# Autodesk Inventor assembly: 043-DP
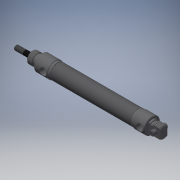
[picture p0: Inventor's stored thumbnail of the model, 180x180]
Saved by Autodesk Inventor 2016 (Build 200138000, 138)
## iProperties
Category: PARTsolutions
Company: BIMBA
Created: 2016-01-18
Part Number: 043-DP
Catalog Web Link: www.cadenas.de
Description: Original Line Standard Air Cylinders-
Vendor: BIMBA
Document SubType Name: Assembly
Designer: psAdmin
Manufacturer: BIMBA
PSOL_IDENT_0: {$CADENAS_DATA\23d-libs\bimba\bimba\bimba_imperial\bimba_full_line\original_line_cylinders\standard_
PSOL_IDENT_1: air_cylinders\standard_air_cylinder_asmtab.prj},312 {VTYP=3D},{STYP=ASSTAB},{NB=043-DP},{LINA=043-DP
PSOL_IDENT_2: },{NN=Original Line Standard Air Cylinders},{DATE=02.12.2015 13:51:22},{GEOMDATE=02.12.2015 13:51:20
PSOL_IDENT_3: },{VERSION=},{LINEID=50},{LINESUBID=-1},{WBVAR=STROKE,ACTING,MNT,DER,NR,BM,CO,OO,VO,M,EE,EEL,K,Q,Y,G
PSOL_IDENT_4: ,T,B,H,SER,SR,NT,W,HL,STPT1,STPT2,STPT3,STPT4,MB,PB,PRC,TB,MN}  {NB=043-DP},{LINA=043-DP},{KT=DUMMY}
PSOL_IDENT_5: ,{PN=043-DP},{PNC=043-DP},{PNA=(NO ACCESSORIES)},{DASH=-},{BORE1=0.75000000},{BORE=3/4\" (04)},{BORE
PSOL_IDENT_6: PN=04},{STROKE=3.000},{STROKEALG=[0.011:50/0.001]},{STROKE1=3.000},{ACTING=D},{ACTINGALG= '' , 'Sing
PSOL_IDENT_7: le Acting (SA)' , 'R' , 'Reverse Single Acting (SA)' , 'D' , 'Double Acting (SA)' },{ACTINGPN=D},{MN
PSOL_IDENT_8: T=P},{MNTALG= '' , 'Front Nose Mounting (SA)' , 'P' , 'Rear Pivot Mounting (SA)' , 'XP' , 'Double En
PSOL_IDENT_9: d or Pivot Mounting (SA)' , 'X' , 'Double End Mounting (SA)' , 'BF' , 'Front Block Mounting (SA)' , '
PSOL_IDENT_10: BR' , 'Rear Block Mounting for Vertical Positioning (SA)' , 'BFT' , 'Front Block Trunnion Mounting (
PSOL_IDENT_11: SA)' , 'BRT' , 'Rear Block Trunnion Mounting (SA)' },{TYPE=},{MNTPN=P},{DER=},{DERALG= '' , 'N/A' },
PSOL_IDENT_12: {NR=},{NRALG= '' , 'N/A' },{NRPN=},{BM=},{BMALG= '' , 'N/A' },{BMPN=},{CO=},{COALG= '' , 'N/A' },{OO=
PSOL_IDENT_13: },{OOALG= '', 'N/A' },{OOPN=},{VO=Z},{VOALG= 'Z' , 'N/A' },{VOPN=},{OOVOPN=},{M=},{MALG= '', 'Withou
PSOL_IDENT_14: t Magnet', 'M', 'With Magnet' },{EE=},{EEL=0.000},{EEMAX=47.0000},{EEALG= '', 'Without Extra Extensi
PSOL_IDENT_15: on', 'EE', 'With Extra Extension' },{EELALG=0},{EEPN=},{EEPN1=0.000},{K=},{KALG= '', 'Standard' , 'K'
PSOL_IDENT_16: , 'Ports Rotated 90deg K' },{KPN=},{Q=},{QALG= '' , 'N/A' },{QPN=},{Y=},{YALG= '' , 'Without Pivot
PSOL_IDENT_17: Bushing' , 'Y' , 'With Pivot Bushing' },{YPN=},{YCON=},{F=},{FALG= '', 'Non-Coated (Standard)', 'F',
PSOL_IDENT_18: 'Molycoated' },{FPN=},{G=},{GPN=},{GPN99=},{T=},{TALG= '' , 'Standard -20° to 200°F (-29° to 95°C)'
PSOL_IDENT_19: , 'N' , 'Low Temperature' , 'V' , 'High Temperature' },{NPN=},{VPN=},{B=},{BALG= '', 'W/out Bumpers'
PSOL_IDENT_20: , 'B' , 'W/ Bumpers' },{BPN=},{H=},{HALG= '', 'N/A' },{HPN=},{SER=},{SERALG= '' , 'Without Spring E
PSOL_IDENT_21: xtend/Return' , 'JS' , 'With Spring Return' , 'JR' , 'With Spring Extend' },{SR=C},{SRALG= 'C' , 'St
PSOL_IDENT_22: andard Blackened Carbon Steel' , 'SR' , 'Stainless Steel [SR]' },{SRPN=},{SRCON=1},{NT=},{NTPN=},{W=
PSOL_IDENT_23: },{WALG= '' , 'Without Wiper' , 'W' , 'With Wiper' },{WPN=},{E=},{EALG= '' , 'Standard Seals/Lube' ,
PSOL_IDENT_24: 'E' , 'Non-Lube Seals/Lube' },{EPN=},{HL=},{HLALG= '' , 'Without Low Pressure Hydraulic' , 'HL' , '
PSOL_IDENT_25: With Low Pressure Hydraulic' },{ST=},{STALG= '' , 'N/A' },{STPT1=},{STPT1ALG= '' , 'N/A' },{STPT2=},
PSOL_IDENT_26: {STPT2ALG= '' , 'N/A' },{STPT3=},{STPT3ALG= '' , 'N/A' },{STPT4=},{STPT4ALG= '' , 'N/A' },{STPN=},{M
PSOL_IDENT_27: B=},{MBALG= '' , 'N/A' },{MBPN=},{MBPNALL=},{MBPNALLREAR=},{PB=},{PBALG= '' , 'Without Pivot Bracket'
PSOL_IDENT_28: , 'D-167' , 'D-167' },{PBPN=},{PBPNALL=D-167},{PRC=},{PRCALG= '' , 'W/out Pivot Rod Clevis' , 'F,D-
PSOL_IDENT_29: 166-3' , 'D-166-3 (front)' },{PRCPN=},{PRCPNALL=D-166-3},{TB=},{TBALG= '' , 'N/A' },{TBPN=},{TBPNALL=
PSOL_IDENT_30: },{MN=},{MNALG= '' , 'Without Mounting Nut' , 'F,D-9' , 'D-9 (front)' , 'R,D-9' , 'D-9 (rear)', '2x,
PSOL_IDENT_31: D-9' , 'D-9 (front & rear)' },{MNPN=},{MNCONF=},{MNCONR=},{TLEN=4.2555},{FRAC=14.7500},{RGCON=},{RGD
PSOL_IDENT_32: ACCON=R},{RHCON=P},{RHCON1=P},{RHCONON=1},{RHACCON=},{FNUTCON=0},{RNUTCON=0},{FNUTPN=D-9},{RNUTPN=D-
PSOL_IDENT_33: 9},{FNUTTRANS=0.0000},{RNUTTRANS=0.0000},{VHOLECON=0},{A1=1.5940},{A1N=0.8750},{A1P=1.5940},{A1B=1.5
PSOL_IDENT_34: 940},{A4=0.2525},{A4N=0.3130},{A4P=0.2525},{A5=0.0300},{A1H=1.594},{A1NH=0.5310},{A1PH=1.5940},{A1BH=
PSOL_IDENT_35: 1.0940},{A1SH=1.2190},{A2H=0.2190},{A2NH=0.2190},{LENGTH=3.7500},{LENGTH1=3.7500},{LENGTH2=3.8100},{
PSOL_IDENT_36: MUL=3.0000},{MUL11=3.0000},{MUL22=8.07},{MUL33=5.0700},{MUL2=3.0000},{MUL211=3.0000},{MUL222=2.6900}
PSOL_IDENT_37: ,{MUL233=1.6900},{SSS=6.0000},{RGLEN=1.3715},{RHLEN=1.1230},{SSS1=4.0000},{A13=1.3120},{DIF=0.0000},
PSOL_IDENT_38: {G5=0.6250},{ON=0},{SSADD=0.0000},{BADD=0.0000},{MADD=0.0000},{NVADD=0.0000},{TRACKL=3.9655},{TRACKC
PSOL_IDENT_39: ON=D-74168},{TRIMCON=0},{TRIMCON1=0},{PINCON=D-51},{FSPACE=0.5662},{SPACE=0.0750},{TEXT=0.1312},{S1=
PSOL_IDENT_40: 1.0000},{D1=0.8325},{D1N=0.8050},{D1B=0.8625},{D1P=0.8325},{FA=0.940},{RA=0.9400},{PPATH=standard_ai
PSOL_IDENT_41: r_cylinder_asmtpl.prj},{MATALGHTML=<b>Standard Original Line:</b><dl><dt>Rod:</dt><dd>- Stainless St
PSOL_IDENT_42: eel</dd><dd>&nbsp;&nbsp;(5/16 9/16 Bores)</dd><dd>- High Strength Carbon Steel</dd><dd>&nbsp;&nbsp;(
PSOL_IDENT_43: 3/4 3 Bore)</dd><dd>- Stainless Steel</dd><dd>&nbsp;&nbsp;(X style DXP/DX/DXDE)</dd><dt>Bearings:</d
PSOL_IDENT_44: t><dd>- Sintered Bronze</dd><dt>Body:</dt><dd>- 304 Stainless Steel</dd><dt>End Caps:</dt><dd>- Alum
PSOL_IDENT_45: inum</dd><dt>Seals:</dt><dd>- Buna N</dd></dl>},{ASSCFGPRA=04DP},{MBPNA=},{MNPNA=},{PRCPNA=},{ASSOPT
PSOL_IDENT_46: ACC=STPT4},{A=6.75},{HADD=0.0000},{WFL=0.25},{QADD=0.000},{QADD1=0.440},{TEST=3.0000},{MNTB=},{STDNU
PSOL_IDENT_47: TF=0},{STDNUTR=0},{STRK2D=0},{X2D=2},{STROKESW=3.000},{EESW=0.000},{FCD=0},{BCD=0},{RCD=0},{CUSTADD=
PSOL_IDENT_48: 2.000},{FT=1/4-26 UNF-2A},{FT1=1/4-26 UNF-2A},{FT2=5/8-18 UNF-2A},{PORT=1/8 NPT},{FT11=1/2-20 UNF-2A
PSOL_IDENT_49: },{FT12=5/8-18 UNF-2A}
NN: Original Line Standard Air Cylinders
NT: Standard Male Thread
NB: 043-DP
NBSYN: $PNC.
LINA: 043-DP
PN: 043-DP
PNA: (NO ACCESSORIES)
BORE: 3/4" [04]
STROKE: 3.000
ACTING: Double [D]
MNT: Rear Pivot [P]
DER: N/A
NR: N/A
BM: N/A
CO: N/A
OO: N/A
VO: N/A
M: Without Magnet Piston
EE: Standard Rod Extension
EEL: 0.000
K: Standard
Q: N/A
Y: Standard Pivot Style
G: Standard Grease Lube
T: Standard -20° to 200°F (-29° to 95°C)
B: Without Bumpers
H: N/A
SER: Without Failsafe Spring Extend/Return
SR: Standard Blackened Carbon Steel
W: Without Wiper
HL: Standard 250 PSI Air
STPT1: N/A
STPT2: N/A
STPT3: N/A
STPT4: N/A
MB: N/A
PB: Without Pivot Bracket
PRC: Without Piston Rod Clevis
TB: N/A
MN: Without Mounting Nut
A: 6.75
SUPPLIER: BIMBA
ARTICLENO: 043-DP
BOMINFO: 043-DP
CREATOR: CADENAS GmbH
Title: 043-DP
Author: Cadenas PARTsolutions
## Documents named in this file (7)
- C:\Users\Evan\Documents\Inventor\FRC2016\GrabCad\Imported Components\Cylinders\Cylinders\0.75x3 adaptive\043-DP.iam
- C:\Users\Evan\Documents\Inventor\FRC2016\GrabCad\Imported Components\Cylinders\Cylinders\0.75x3 adaptive\043-DPC0000_0_dummy.ipt
- C:\Users\Evan\Documents\Inventor\FRC2016\GrabCad\Imported Components\Cylinders\Cylinders\0.75x3 adaptive\04R000-0_rod_guide.ipt
- C:\Users\Evan\Documents\Inventor\FRC2016\GrabCad\Imported Components\Cylinders\Cylinders\0.75x3 adaptive\04R-4_25550C.ipt
- C:\Users\Evan\Documents\Inventor\FRC2016\GrabCad\Imported Components\Cylinders\Cylinders\0.75x3 adaptive\04P0000_rear_head.ipt
- C:\Users\Evan\Documents\Inventor\FRC2016\GrabCad\Imported Components\Cylinders\Cylinders\0.75x3 adaptive\D-51.ipt
- C:\Users\Evan\Documents\Inventor\FRC2016\GrabCad\Imported Components\Cylinders\Cylinders\0.75x3 adaptive\C-043-DP0_rod.ipt
## Components (6 placed, 6 different names)
1. 043-DPC0000_0_dummy:1
2. 04R000-0_rod_guide:1
3. 04R-4_25550C:1 — Mate:1
4. 04P0000_rear_head:1
5. D-51:1
6. C-043-DP0_rod:1 — Mate:1
## Relationships (1: Mate 1)
- Mate:1: 04R-4_25550C:1 ↔ C-043-DP0_rod:1
